# Autodesk Inventor assembly: Penholder
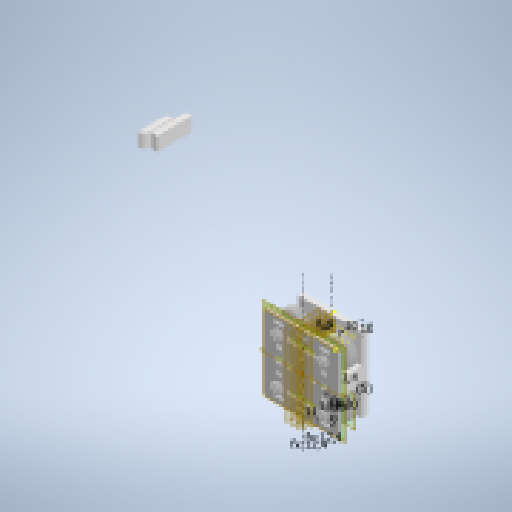
[picture p0: Inventor's stored thumbnail of the model, 512x512]
Saved by Autodesk Inventor 2023 (Build 270158000, 158)
## iProperties
Created: 2023-08-18
Part Number: Penholder
Document SubType Name: Assembly
Designer: Felix
Author: Felix
## Documents named in this file (6)
- D:\Programmieren\PineapplePenPlotter\Inventor\try_3\Penholder.iam
- D:\Programmieren\PineapplePenPlotter\Inventor\try_3\BeltClamp.ipt
- D:\Programmieren\PineapplePenPlotter\Inventor\try_3\Penholder\Frontside.ipt
- D:\Programmieren\PineapplePenPlotter\Inventor\StoreBought\4022_20220624140806_V-Slot Gantry Kit - 20mm.iam
- D:\Programmieren\PineapplePenPlotter\Inventor\try_3\Penholder\Backside.ipt
- D:\Programmieren\PineapplePenPlotter\Inventor\try_3\BeltClampTensioner.ipt
## Components (5 placed, 5 different names)
1. BeltClamp:2
2. Frontside:1
3. 4022_20220624140806_V-Slot Gantry Kit - 20mm:1 [sub-assembly] — Flush:1, Flush:3, Flush:4, Mate:1, Angle:1, Flush:7
4. Backside:1 — Flush:3, Flush:4, Flush:7, Flush:8
5. BeltClampTensioner:1
## Relationships (9: Flush 7, Mate 1, Angle 1)
- Flush:1 (-11 mm): 4022_20220624140806_V-Slot Gantry Kit - 20mm:1
- Flush:3: 4022_20220624140806_V-Slot Gantry Kit - 20mm:1 ↔ Backside:1
- Flush:4: 4022_20220624140806_V-Slot Gantry Kit - 20mm:1 ↔ Backside:1
- Mate:1: 4022_20220624140806_V-Slot Gantry Kit - 20mm:1
- Angle:1 (0 deg): 4022_20220624140806_V-Slot Gantry Kit - 20mm:1
- Flush:5 (3.95 mm)
- Flush:6 (-5.05 mm)
- Flush:7: 4022_20220624140806_V-Slot Gantry Kit - 20mm:1 ↔ Backside:1
- Flush:8: Backside:1
